# Autodesk Inventor assembly: lw_6_сборка3
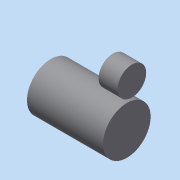
[picture p0: Inventor's stored thumbnail of the model, 180x180]
Saved by Autodesk Inventor 2019 (Build 230136000, 136)
## iProperties
Created: 2021-05-14
Part Number: lw_6_сборка3
Material: Типовые
Document SubType Name: Assembly
Designer: Kurbatova
Author: Kurbatova
## Documents named in this file (3)
- C:\Users\Kurbatova\source\LW2021\LW_SAPR\Сборки\lw_6_сборка3.iam
- C:\Users\Kurbatova\source\LW2021\LW_SAPR\Детали\lw_6_part3_cilindr1.ipt
- C:\Users\Kurbatova\source\LW2021\LW_SAPR\Детали\lw_6_part3_wheel.ipt
## Components (2 placed, 2 different names)
1. lw_6_part3_cilindr1:1 — Угол:1
2. lw_6_part3_wheel:1 — Угол:1
## Relationships (1: Angle 1)
- Угол:1 [Angle] (90 deg): lw_6_part3_cilindr1:1 ↔ lw_6_part3_wheel:1
